# Autodesk Inventor assembly: Camera
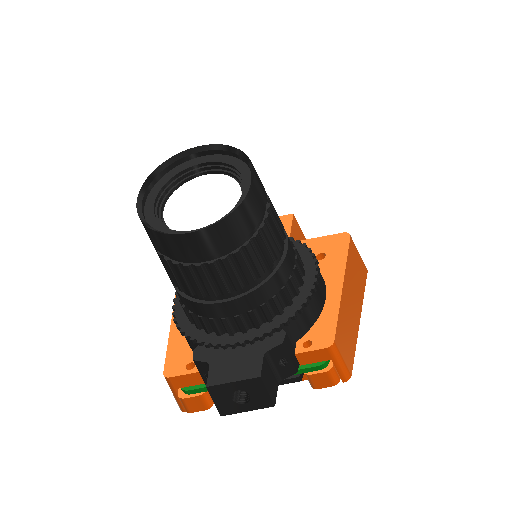
[picture p0: Inventor's stored thumbnail of the model, 512x512]
Saved by Autodesk Inventor 2025.2 (Build 292293000, 293)
## iProperties
Created: 2026-05-17
Part Number: Camera
Document SubType Name: Assembly
Designer: rolan
Author: rolan
## Documents named in this file (4)
- C:\Users\rolan\Documents\PhD\Inventor\Assembly\Camera.iam
- C:\Users\rolan\Documents\PhD\Inventor\Parts\CameraMountFront.ipt
- C:\Users\rolan\Documents\PhD\Inventor\3D Files\Raspberry Pi HQ Camera with cs mount lens v3\Raspberry Pi HQ Camera with cs mount lens v3\Raspberry Pi HQ Camera with cs mount lens v3.ipt
- C:\Users\rolan\Documents\PhD\Inventor\Parts\CameraMountBack.ipt
## Components (3 placed, 3 different names)
1. CameraMountFront:1 — Mate:1, Mate:2, Mate:3
2. Raspberry Pi HQ Camera with cs mount lens v3:1 — Mate:1, Mate:2, Mate:3, Mate:4, Mate:5, Mate:6
3. CameraMountBack:1 — Mate:4, Mate:5, Mate:6
## Relationships (6: Mate 6)
- Mate:1: CameraMountFront:1 ↔ Raspberry Pi HQ Camera with cs mount lens v3:1
- Mate:2: CameraMountFront:1 ↔ Raspberry Pi HQ Camera with cs mount lens v3:1
- Mate:3: CameraMountFront:1 ↔ Raspberry Pi HQ Camera with cs mount lens v3:1
- Mate:4: Raspberry Pi HQ Camera with cs mount lens v3:1 ↔ CameraMountBack:1
- Mate:5: Raspberry Pi HQ Camera with cs mount lens v3:1 ↔ CameraMountBack:1
- Mate:6: Raspberry Pi HQ Camera with cs mount lens v3:1 ↔ CameraMountBack:1
